# Autodesk Inventor assembly: POM_T5_11
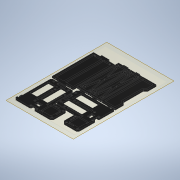
[picture p0: Inventor's stored thumbnail of the model, 180x180]
Saved by Autodesk Inventor 2020 (Build 240168000, 168)
## iProperties
Created: 2021-08-27
Part Number: POM_T5_11
Document SubType Name: Assembly
Designer: Masato
Author: Masato
## Documents named in this file (8)
- C:\Users\naoki\Documents\Inventor\CitBrains\git_clone\OpenPlatform4_1\コックピット\OpenPlatform_ver3_0\cam\POM_T5_11.iam
- C:\Users\naoki\Documents\Inventor\CitBrains\git_clone\OpenPlatform4_1\コックピット\OpenPlatform_ver3_0\cam\Disposable_Board.ipt
- C:\Users\naoki\Documents\Inventor\CitBrains\git_clone\OpenPlatform4_1\コックピット\OpenPlatform_ver3_0\UpperBody\Cockpit\Cockpit_battery_back_boor.ipt
- C:\Users\naoki\Documents\Inventor\CitBrains\git_clone\OpenPlatform4_1\コックピット\OpenPlatform_ver3_0\UpperBody\Cockpit\Cockpit_battery_bottom_frame.ipt
- C:\Users\naoki\Documents\Inventor\CitBrains\git_clone\OpenPlatform4_1\コックピット\OpenPlatform_ver3_0\UpperBody\Cockpit\Cockpit_battery_front_frame.ipt
- C:\Users\naoki\Documents\Inventor\CitBrains\git_clone\OpenPlatform4_1\コックピット\OpenPlatform_ver3_0\UpperBody\Cockpit\Cockpit_front_frame.ipt
- C:\Users\naoki\Documents\Inventor\CitBrains\git_clone\OpenPlatform4_1\コックピット\OpenPlatform_ver3_0\UpperBody\Cockpit\Cockpit_side_frame.ipt
- C:\Users\naoki\Documents\Inventor\CitBrains\git_clone\OpenPlatform4_1\コックピット\OpenPlatform_ver3_0\UpperBody\Cockpit\Cockpit_side_frame_MIR.ipt
## Components (7 placed, 7 different names)
1. Disposable_Board:1 — メイト:2, メイト:1, フラッシュ:1, フラッシュ:2, メイト:4, メイト:5, メイト:6, メイト:7, メイト:8, メイト:9, フラッシュ:3, フラッシュ:4, フラッシュ:5
2. Cockpit_battery_back_boor:1 — メイト:8, メイト:20, メイト:25, メイト:26
3. Cockpit_battery_bottom_frame:1 — メイト:9, メイト:21, メイト:22, メイト:23
4. Cockpit_battery_front_frame:1 — メイト:6, メイト:23, メイト:24, メイト:25
5. Cockpit_front_frame:1 — メイト:7, メイト:15, フラッシュ:5, メイト:22
6. Cockpit_side_frame:1 — メイト:4, メイト:13, メイト:14, メイト:20, メイト:21, メイト:24, メイト:26
7. Cockpit_side_frame_MIR:1 — メイト:5, フラッシュ:3, フラッシュ:4, メイト:13, メイト:14, メイト:15
## Relationships (23: Mate 18, Flush 5)
- メイト:2 [Mate]: Disposable_Board:1
- メイト:1 [Mate]: Disposable_Board:1
- フラッシュ:1 [Flush]: Disposable_Board:1
- フラッシュ:2 [Flush]: Disposable_Board:1
- メイト:4 [Mate]: Disposable_Board:1 ↔ Cockpit_side_frame:1
- メイト:5 [Mate]: Disposable_Board:1 ↔ Cockpit_side_frame_MIR:1
- メイト:6 [Mate]: Disposable_Board:1 ↔ Cockpit_battery_front_frame:1
- メイト:7 [Mate]: Disposable_Board:1 ↔ Cockpit_front_frame:1
- メイト:8 [Mate]: Disposable_Board:1 ↔ Cockpit_battery_back_boor:1
- メイト:9 [Mate]: Disposable_Board:1 ↔ Cockpit_battery_bottom_frame:1
- フラッシュ:3 [Flush] (2 mm): Disposable_Board:1 ↔ Cockpit_side_frame_MIR:1
- フラッシュ:4 [Flush] (2 mm): Disposable_Board:1 ↔ Cockpit_side_frame_MIR:1
- メイト:13 [Mate] (2.5 mm): Cockpit_side_frame:1 ↔ Cockpit_side_frame_MIR:1
- メイト:14 [Mate] (2.5 mm): Cockpit_side_frame:1 ↔ Cockpit_side_frame_MIR:1
- メイト:15 [Mate] (2.5 mm): Cockpit_front_frame:1 ↔ Cockpit_side_frame_MIR:1
- フラッシュ:5 [Flush] (2 mm): Disposable_Board:1 ↔ Cockpit_front_frame:1
- メイト:20 [Mate] (2.5 mm): Cockpit_battery_back_boor:1 ↔ Cockpit_side_frame:1
- メイト:21 [Mate] (2.5 mm): Cockpit_battery_bottom_frame:1 ↔ Cockpit_side_frame:1
- メイト:22 [Mate] (2.5 mm): Cockpit_battery_bottom_frame:1 ↔ Cockpit_front_frame:1
- メイト:23 [Mate] (2.5 mm): Cockpit_battery_bottom_frame:1 ↔ Cockpit_battery_front_frame:1
- メイト:24 [Mate] (2.5 mm): Cockpit_battery_front_frame:1 ↔ Cockpit_side_frame:1
- メイト:25 [Mate] (2.5 mm): Cockpit_battery_back_boor:1 ↔ Cockpit_battery_front_frame:1
- メイト:26 [Mate] (2.5 mm): Cockpit_battery_back_boor:1 ↔ Cockpit_side_frame:1
